# Autodesk Inventor assembly: caja_pedalera
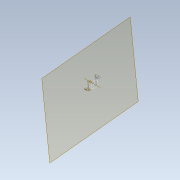
[picture p0: Inventor's stored thumbnail of the model, 180x180]
Saved by Autodesk Inventor 2021 (Build 250183000, 183)
## iProperties
Created: 2021-04-24
Part Number: caja_pedalera
Document SubType Name: Assembly
Designer: j2seb
Author: j2seb
## Documents named in this file (10)
- G:\Unidades compartidas\APM\02 Inventor-Drive\caja_pedalera.iam
- G:\Unidades compartidas\APM\02 Inventor-Drive\cazoleta.ipt
- G:\Unidades compartidas\APM\02 Inventor-Drive\centro.ipt
- G:\Unidades compartidas\APM\02 Inventor-Drive\balines.ipt
- G:\Unidades compartidas\APM\02 Inventor-Drive\tapa casoleta.ipt
- G:\Unidades compartidas\APM\02 Inventor-Drive\arandela.ipt
- G:\Unidades compartidas\APM\02 Inventor-Drive\tuerca.ipt
- G:\Unidades compartidas\APM\02 Inventor-Drive\Ensamblaje pedal.iam
- C:\Users\j2seb\OneDrive\Documents\Inventor\Content Center Files\R2021\es-ES\DIN 439-2\DIN 439 - M16 x 1,5.ipt
- G:\Unidades compartidas\APM\02 Inventor-Drive\Transmision\Design Accelerator\Roller Chain Sprocket21.ipt
## Components (16 placed, 9 different names)
1. cazoleta:1 — Coincidencia:1, Coincidencia:2, Nivelación:1, Nivelación:3
2. cazoleta:2 — Coincidencia:3, Coincidencia:4, Coincidencia:8, Nivelación:2
3. centro:1 — Coincidencia:5, Coincidencia:6, Coincidencia:7, Coincidencia:9, Coincidencia:10, Coincidencia:11, Coincidencia:12, Coincidencia:15, Coincidencia:16, Coincidencia:19, Coincidencia:20, Coincidencia:21, Coincidencia:22, Nivelación:4, Coincidencia:24, Coincidencia:26, Coincidencia:27, Coincidencia:28
4. balines:1 — Coincidencia:6, Nivelación:1
5. balines:2 — Coincidencia:7, Coincidencia:8
6. tapa casoleta:1 — Coincidencia:9, Nivelación:3, Coincidencia:13
7. tapa casoleta:2 — Coincidencia:10, Nivelación:2, Coincidencia:14
8. arandela:1 — Coincidencia:11, Coincidencia:14, Coincidencia:17
9. arandela:2 — Coincidencia:12, Coincidencia:13, Coincidencia:18
10. tuerca:1 — Coincidencia:15, Coincidencia:17
11. tuerca:2 — Coincidencia:16, Coincidencia:18
12. Ensamblaje pedal:1 [sub-assembly] — Coincidencia:19, Coincidencia:20, Coincidencia:25
13. Ensamblaje pedal:2 [sub-assembly] — Coincidencia:21, Coincidencia:22, Coincidencia:23
14. DIN 439-2 - reemplazado por DIN EN 24035/28675 M16 x 1,5:1 — Coincidencia:23, Coincidencia:24
15. DIN 439-2 - reemplazado por DIN EN 24035/28675 M16 x 1,5:2 — Coincidencia:25, Coincidencia:26
16. Roller Chain Sprocket2:1 — Coincidencia:27, Coincidencia:28
## Relationships (32: Mate 28, Flush 4)
- Coincidencia:1 [Mate]: cazoleta:1
- Coincidencia:2 [Mate] (-36 mm): cazoleta:1
- Coincidencia:3 [Mate]: cazoleta:2
- Coincidencia:4 [Mate] (-36 mm): cazoleta:2
- Coincidencia:5 [Mate]: centro:1
- Coincidencia:6 [Mate]: centro:1 ↔ balines:1
- Coincidencia:7 [Mate]: centro:1 ↔ balines:2
- Coincidencia:8 [Mate] (-8 mm): cazoleta:2 ↔ balines:2
- Nivelación:1 [Flush] (-8 mm): cazoleta:1 ↔ balines:1
- Coincidencia:9 [Mate]: centro:1 ↔ tapa casoleta:1
- Coincidencia:10 [Mate]: centro:1 ↔ tapa casoleta:2
- Nivelación:2 [Flush]: cazoleta:2 ↔ tapa casoleta:2
- Nivelación:3 [Flush]: cazoleta:1 ↔ tapa casoleta:1
- Coincidencia:11 [Mate]: centro:1 ↔ arandela:1
- Coincidencia:12 [Mate]: centro:1 ↔ arandela:2
- Coincidencia:13 [Mate]: tapa casoleta:1 ↔ arandela:2
- Coincidencia:14 [Mate]: tapa casoleta:2 ↔ arandela:1
- Coincidencia:15 [Mate]: centro:1 ↔ tuerca:1
- Coincidencia:16 [Mate]: centro:1 ↔ tuerca:2
- Coincidencia:17 [Mate]: arandela:1 ↔ tuerca:1
- Coincidencia:18 [Mate]: arandela:2 ↔ tuerca:2
- Coincidencia:19 [Mate]: centro:1 ↔ Ensamblaje pedal:1
- Coincidencia:20 [Mate]: centro:1 ↔ Ensamblaje pedal:1
- Coincidencia:21 [Mate]: centro:1 ↔ Ensamblaje pedal:2
- Coincidencia:22 [Mate]: centro:1 ↔ Ensamblaje pedal:2
- Nivelación:4 [Flush]: centro:1
- Coincidencia:23 [Mate]: Ensamblaje pedal:2 ↔ DIN 439-2 - reemplazado por DIN EN 24035/28675 M16 x 1,5:1
- Coincidencia:24 [Mate]: centro:1 ↔ DIN 439-2 - reemplazado por DIN EN 24035/28675 M16 x 1,5:1
- Coincidencia:25 [Mate]: Ensamblaje pedal:1 ↔ DIN 439-2 - reemplazado por DIN EN 24035/28675 M16 x 1,5:2
- Coincidencia:26 [Mate]: centro:1 ↔ DIN 439-2 - reemplazado por DIN EN 24035/28675 M16 x 1,5:2
- Coincidencia:27 [Mate]: centro:1 ↔ Roller Chain Sprocket2:1
- Coincidencia:28 [Mate] (50 mm): centro:1 ↔ Roller Chain Sprocket2:1
## Named parameters: long = 72 mm
